# Autodesk Inventor assembly: SEA Gearbox
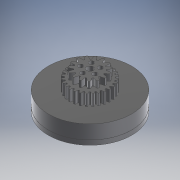
[picture p0: Inventor's stored thumbnail of the model, 180x180]
Saved by Autodesk Inventor 2017 SP1 (Build 210196100, 196)
## iProperties
Created: 2019-09-07
Part Number: SEA Gearbox
Document SubType Name: Assembly
Designer: Dell
Author: Dell
## Documents named in this file (5)
- C:\Users\Zach\Documents\GitHub\tr2\Actuator 1.5\SEA Gearbox.iam
- C:\Users\Zach\Documents\GitHub\tr2\Actuator 1.5\SE01.ipt
- C:\Users\Zach\Documents\GitHub\tr2\Actuator 1.5\SE02.ipt
- C:\Users\Zach\Documents\GitHub\tr2\Actuator 1.5\SE03.ipt
- C:\Users\Zach\Documents\GitHub\tr2\Actuator 1.5\SEA Gearbox\Design Accelerator\Spur Gears3.iam
## Components (4 placed, 4 different names)
1. SE01:1 — Mate:5, Mate:7, Mate:8, Mate:9
2. SE02:1 — Mate:7, Angle:1, Mate:8, Mate:12, Mate:13, Mate:14
3. SE03:1 — Mate:5, Angle:1, Mate:9
4. Spur Gears:1 [sub-assembly] — Mate:12, Mate:13, Mate:14
## Relationships (8: Mate 7, Angle 1)
- Mate:5: SE01:1 ↔ SE03:1
- Mate:7: SE01:1 ↔ SE02:1
- Angle:1 (180 deg): SE02:1 ↔ SE03:1
- Mate:8: SE01:1 ↔ SE02:1
- Mate:9: SE01:1 ↔ SE03:1
- Mate:12: SE02:1 ↔ Spur Gears:1
- Mate:13: SE02:1 ↔ Spur Gears:1
- Mate:14: SE02:1 ↔ Spur Gears:1
